# Autodesk Inventor assembly: Desk Assembly
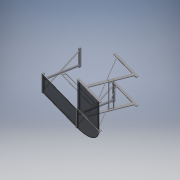
[picture p0: Inventor's stored thumbnail of the model, 180x180]
Saved by Autodesk Inventor 2016 (Build 200138000, 138)
## iProperties
Created: 2015-11-20
Part Number: Desk Assembly
Material: 常规
Document SubType Name: Assembly
Designer: Shawn Shi Feng
Author: Shawn Shi Feng
## Documents named in this file (8)
- E:\Black glass top desk\Desk Assembly.iam
- E:\Black glass top desk\Black Glass Corner Piece.ipt
- E:\Black glass top desk\Black Glass Piece.ipt
- E:\Black glass top desk\Desk stand.ipt
- E:\Black glass top desk\Desk foot holding bar.ipt
- E:\Black glass top desk\Desk glass holding bar.ipt
- E:\Black glass top desk\Hex Screws used in Desk.ipt
- E:\Black glass top desk\Corner glass holding bar.ipt
## Components (30 placed, 7 different names)
1. Black Glass Corner Piece:1 — 配合:15, 配合:16
2. Black Glass Piece:1 — Mate:22, Mate:23, Mate:24, Mate:25
3. Black Glass Piece:2 — Mate:18, Mate:19, Mate:20, Mate:21
4. Desk stand:1 — 配合:2, 角度:1, 插入:37, 插入:38, 配合:17, 插入:39, 插入:44, 插入:45, Mate:23
5. Desk stand:2 — 插入:11, 插入:12, 插入:15, 插入:16, 插入:23, 插入:26, 角度:4, 插入:29, 插入:30, Mate:18
6. Desk stand:3 — 插入:13, 插入:14, 插入:17, 插入:18, 插入:24, 插入:25, 角度:5, 插入:33, 插入:34, Mate:19
7. Desk stand:4 — 插入:5, 插入:6, 插入:7, 插入:8, 配合:6, 角度:3, 插入:40, 插入:41, 插入:42, 插入:43, Mate:22
8. Desk foot holding bar:1 — 配合:2, 插入:7, 插入:8
9. Desk foot holding bar:2 — 插入:15, 插入:16, 插入:17, 插入:18
10. Desk glass holding bar:1 — 角度:1, 插入:39, 插入:43, Mate:24
11. Desk glass holding bar:2 — 配合:6, 角度:3, 配合:17, 插入:41, Mate:25
12. Desk glass holding bar:3 — 插入:23, 插入:24, 角度:5, Mate:21
13. Desk glass holding bar:4 — 插入:25, 插入:26, 角度:4, Mate:20
14. Hex Screws used in Desk:1 — 插入:11
15. Hex Screws used in Desk:2 — 插入:12
16. Hex Screws used in Desk:3 — 插入:5
17. Hex Screws used in Desk:4 — 插入:42
18. Hex Screws used in Desk:5 — 插入:6
19. Hex Screws used in Desk:6 — 插入:14
20. Hex Screws used in Desk:7 — 插入:13
21. Hex Screws used in Desk:8 — 插入:40
22. Hex Screws used in Desk:9 — 插入:30
23. Hex Screws used in Desk:10 — 插入:29
24. Hex Screws used in Desk:11 — 插入:31
25. Hex Screws used in Desk:12 — 插入:32
26. Corner glass holding bar:1 — 插入:31, 插入:32, 插入:33, 插入:34, 插入:35, 插入:36, 插入:37, 插入:38, 配合:15, 配合:16
27. Hex Screws used in Desk:13 — 插入:45
28. Hex Screws used in Desk:14 — 插入:36
29. Hex Screws used in Desk:15 — 插入:44
30. Hex Screws used in Desk:16 — 插入:35
## Relationships (50: Insert 33, Mate 13, Angle 4)
- 配合:2 [Mate]: Desk stand:1 ↔ Desk foot holding bar:1
- 插入:5 [Insert]: Desk stand:4 ↔ Hex Screws used in Desk:3
- 插入:6 [Insert]: Desk stand:4 ↔ Hex Screws used in Desk:5
- 插入:7 [Insert]: Desk stand:4 ↔ Desk foot holding bar:1
- 插入:8 [Insert]: Desk stand:4 ↔ Desk foot holding bar:1
- 角度:1 [Angle] (90 deg): Desk stand:1 ↔ Desk glass holding bar:1
- 配合:6 [Mate]: Desk stand:4 ↔ Desk glass holding bar:2
- 角度:3 [Angle] (90 deg): Desk stand:4 ↔ Desk glass holding bar:2
- 插入:11 [Insert]: Desk stand:2 ↔ Hex Screws used in Desk:1
- 插入:12 [Insert]: Desk stand:2 ↔ Hex Screws used in Desk:2
- 插入:13 [Insert]: Desk stand:3 ↔ Hex Screws used in Desk:7
- 插入:14 [Insert]: Desk stand:3 ↔ Hex Screws used in Desk:6
- 插入:15 [Insert]: Desk stand:2 ↔ Desk foot holding bar:2
- 插入:16 [Insert]: Desk stand:2 ↔ Desk foot holding bar:2
- 插入:17 [Insert]: Desk stand:3 ↔ Desk foot holding bar:2
- 插入:18 [Insert]: Desk stand:3 ↔ Desk foot holding bar:2
- 插入:23 [Insert]: Desk stand:2 ↔ Desk glass holding bar:3
- 插入:24 [Insert]: Desk stand:3 ↔ Desk glass holding bar:3
- 插入:25 [Insert]: Desk stand:3 ↔ Desk glass holding bar:4
- 插入:26 [Insert]: Desk stand:2 ↔ Desk glass holding bar:4
- 角度:4 [Angle] (90 deg): Desk stand:2 ↔ Desk glass holding bar:4
- 角度:5 [Angle] (90 deg): Desk stand:3 ↔ Desk glass holding bar:3
- 插入:29 [Insert]: Desk stand:2 ↔ Hex Screws used in Desk:10
- 插入:30 [Insert]: Desk stand:2 ↔ Hex Screws used in Desk:9
- 插入:31 [Insert]: Hex Screws used in Desk:11 ↔ Corner glass holding bar:1
- 插入:32 [Insert]: Hex Screws used in Desk:12 ↔ Corner glass holding bar:1
- 插入:33 [Insert]: Desk stand:3 ↔ Corner glass holding bar:1
- 插入:34 [Insert]: Desk stand:3 ↔ Corner glass holding bar:1
- 插入:35 [Insert]: Corner glass holding bar:1 ↔ Hex Screws used in Desk:16
- 插入:36 [Insert]: Corner glass holding bar:1 ↔ Hex Screws used in Desk:14
- 插入:37 [Insert]: Desk stand:1 ↔ Corner glass holding bar:1
- 插入:38 [Insert]: Desk stand:1 ↔ Corner glass holding bar:1
- 配合:15 [Mate]: Black Glass Corner Piece:1 ↔ Corner glass holding bar:1
- 配合:16 [Mate]: Black Glass Corner Piece:1 ↔ Corner glass holding bar:1
- 配合:17 [Mate]: Desk stand:1 ↔ Desk glass holding bar:2
- 插入:39 [Insert]: Desk stand:1 ↔ Desk glass holding bar:1
- 插入:40 [Insert]: Desk stand:4 ↔ Hex Screws used in Desk:8
- 插入:41 [Insert]: Desk stand:4 ↔ Desk glass holding bar:2
- 插入:42 [Insert]: Desk stand:4 ↔ Hex Screws used in Desk:4
- 插入:43 [Insert]: Desk stand:4 ↔ Desk glass holding bar:1
- 插入:44 [Insert]: Desk stand:1 ↔ Hex Screws used in Desk:15
- 插入:45 [Insert]: Desk stand:1 ↔ Hex Screws used in Desk:13
- Mate:18: Black Glass Piece:2 ↔ Desk stand:2
- Mate:19: Black Glass Piece:2 ↔ Desk stand:3
- Mate:20: Black Glass Piece:2 ↔ Desk glass holding bar:4
- Mate:21: Black Glass Piece:2 ↔ Desk glass holding bar:3
- Mate:22: Black Glass Piece:1 ↔ Desk stand:4
- Mate:23: Black Glass Piece:1 ↔ Desk stand:1
- Mate:24: Black Glass Piece:1 ↔ Desk glass holding bar:1
- Mate:25: Black Glass Piece:1 ↔ Desk glass holding bar:2
